# Autodesk Inventor assembly: IRB120 plate assy
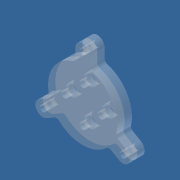
[picture p0: Inventor's stored thumbnail of the model, 180x180]
Saved by Autodesk Inventor 2012 (Build 160160000, 160)
## iProperties
Created: 2013-01-23
Part Number: IRB120 plate assy
Document SubType Name: Assembly
Designer: Edward
Author: Edward
## Documents named in this file (3)
- C:\Users\Edward\Documents\masters\Mechanical\Gripper\IRB120 plate assy.iam
- C:\Users\Edward\Documents\masters\Mechanical\Gripper\acrylic IRB120 plate 2.ipt
- C:\Users\Edward\Documents\masters\Mechanical\Gripper\acrylic IRB120 plate.ipt
## Components (2 placed, 2 different names)
1. acrylic IRB120 plate 2:1 — Insert:1, Insert:2
2. acrylic IRB120 plate:1 — Insert:1, Insert:2
## Relationships (2: Insert 2)
- Insert:1: acrylic IRB120 plate 2:1 ↔ acrylic IRB120 plate:1
- Insert:2: acrylic IRB120 plate 2:1 ↔ acrylic IRB120 plate:1
